# Autodesk Inventor assembly: Patch Panel
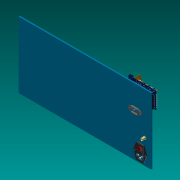
[picture p0: Inventor's stored thumbnail of the model, 180x180]
Saved by Autodesk Inventor 2015 (Build 190159000, 159)
## iProperties
Created: 2015-06-05
Part Number: Patch Panel
Document SubType Name: Assembly
Designer: Sawaiz Syed
Author: Sawaiz Syed
## Documents named in this file (6)
- C:\Users\Admin\SkyDrive\Classes\Reaserch\Black Box\Patch Panel.iam
- C:\Users\Admin\SkyDrive\Classes\Reaserch\Black Box\Imported Components\iec320_703W-00_04\iec320_703W-00_04.ipt
- C:\Users\Admin\SkyDrive\Classes\Reaserch\Black Box\Imported Components\Inlet Module Plug Fuse Switch Male Power Socket 10A 250V 3 Pin IEC320 C14\Inlet Module Plug Fuse Switch Male Power Socket 10A 250V 3 Pin IE.ipt
- C:\Users\Admin\SkyDrive\Classes\Reaserch\Black Box\Imported Components\BNC Coaxial Receptacle - Radiall R141563161\BNC Coaxial Receptacle - Radiall R141563161.iam
- C:\Users\Admin\SkyDrive\Classes\Reaserch\Black Box\Patch Panel.ipt
- C:\Users\Admin\SkyDrive\Classes\Reaserch\Black Box\Imported Components\Gadgets 3D RAMPS 1.4 Complete\Gadgets 3D RAMPS 1.4 Complete.ipt
## Components (5 placed, 5 different names)
1. Patch Panel:1 — Mate:1, Mate:2, Mate:3
2. iec320_703W-00_04:1 — Mate:2
3. Inlet Module Plug Fuse Switch Male Power Socket 10A 250V 3 Pin IE:1 — Mate:1
4. BNC Coaxial Receptacle - Radiall R141563161:1 [sub-assembly] — Mate:3
5. Gadgets 3D RAMPS 1.4 Complete:1
## Relationships (3: Mate 3)
- Mate:1: Patch Panel:1 ↔ Inlet Module Plug Fuse Switch Male Power Socket 10A 250V 3 Pin IE:1
- Mate:2: Patch Panel:1 ↔ iec320_703W-00_04:1
- Mate:3: Patch Panel:1 ↔ BNC Coaxial Receptacle - Radiall R141563161:1
